# Autodesk Inventor assembly: Additional_Building
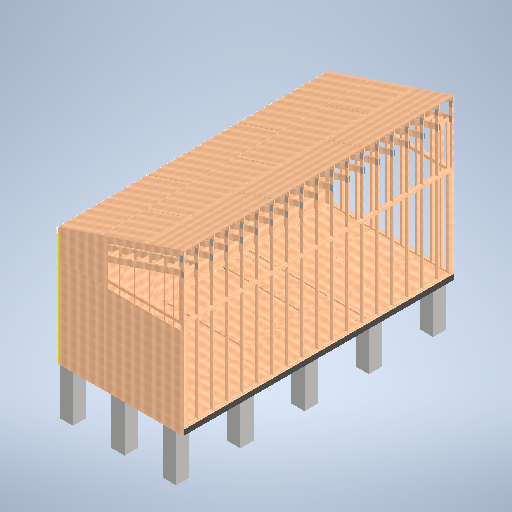
[picture p0: Inventor's stored thumbnail of the model, 512x512]
Saved by Autodesk Inventor 2025 (Build 290162010, 162A)
## iProperties
Created: 2024-08-02
Part Number: Additional_Building
Document SubType Name: Assembly
Designer: Tom
Author: Tom
## Documents named in this file (35)
- C:\Users\Tom\Documents\Inventor\Mobility\Additional_Building\Additional_Building.iam
- C:\Users\Tom\Documents\Inventor\Mobility\Additional_Building\Grid_Of_Piers.iam
- C:\Users\Tom\Documents\Inventor\Mobility\Additional_Building\Floor_System.iam
- C:\Users\Tom\Documents\Inventor\Mobility\Additional_Building\Walls.iam
- C:\Users\Tom\Documents\Inventor\Mobility\Additional_Building\Truss.iam
- C:\Users\Tom\Documents\Inventor\Mobility\Additional_Building\OSB_For_Walls_With_Dimensions_48_x_96_Inches.ipt
- C:\Users\Tom\Documents\Inventor\Mobility\Additional_Building\OSB_For_Walls_With_Dimensions_48_x_48_Inches.ipt
- C:\Users\Tom\Documents\Inventor\Mobility\Additional_Building\OSB_For_Roof_With_Dimensions_96_x_48.ipt
- C:\Users\Tom\Documents\Inventor\Mobility\Additional_Building\OSB_For_Walls_With_Dimensions_25.5_x_96_Inches.ipt
- C:\Users\Tom\Documents\Inventor\Mobility\Additional_Building\Subfascia_With_Width_13.75_Inches.ipt
- C:\Users\Tom\Documents\Inventor\Mobility\Additional_Building\Subfascia_With_Width_14.5_Inches.ipt
- C:\Users\Tom\Documents\Inventor\Mobility\Additional_Building\DensGlass_With_Dimensions_36.5_x_48_Inches.ipt
- C:\Users\Tom\Documents\Inventor\Mobility\Additional_Building\DensGlass_With_Dimensions_48_x_96_Inches.ipt
- C:\Users\Tom\Documents\Inventor\Mobility\Additional_Building\DensGlass_With_Dimensions_48_x_84.5_Inches.ipt
- C:\Users\Tom\Documents\Inventor\Mobility\Additional_Building\DensGlass_With_Dimensions_60.75_x_12_Inches.ipt
- C:\Users\Tom\Documents\Inventor\Mobility\Additional_Building\DensGlass_With_Dimensions_36.5_x_25.5_Inches.ipt
- C:\Users\Tom\Documents\Inventor\Mobility\Additional_Building\DensGlass_With_Dimensions_25.5_x_96_Inches.ipt
- C:\Users\Tom\Documents\Inventor\Mobility\Additional_Building\Siding_For_Back_Wall.iam
- C:\Users\Tom\Documents\Inventor\Mobility\Additional_Building\Fascia.ipt
- C:\Users\Tom\Documents\Inventor\Mobility\Additional_Building\OSB_For_Walls_With_Dimensions_37_x_96_Inches.ipt
- C:\Users\Tom\Documents\Inventor\Mobility\Additional_Building\OSB_For_Side_And_Back.ipt
- C:\Users\Tom\Documents\Inventor\Mobility\Additional_Building\Siding_For_Side_Wall.iam
- C:\Users\Tom\Documents\Inventor\Mobility\Additional_Building\OSB_For_Roof_With_Dimensions_48_x_48.ipt
- C:\Users\Tom\Documents\Inventor\Mobility\Additional_Building\OSB_For_Roof_With_Dimensions_45.796_x_48.ipt
- C:\Users\Tom\Documents\Inventor\Mobility\Additional_Building\Stud_Between_Top_Plate_And_Rafter_1.ipt
- C:\Users\Tom\Documents\Inventor\Mobility\Additional_Building\Stud_Between_Top_Plate_And_Rafter_2.ipt
- C:\Users\Tom\Documents\Inventor\Mobility\Additional_Building\Stud_Between_Top_Plate_And_Rafter_3.ipt
- C:\Users\Tom\Documents\Inventor\Mobility\Additional_Building\Stud_Between_Top_Plate_And_Rafter_4.ipt
- C:\Users\Tom\Documents\Inventor\Mobility\Additional_Building\Stud_Between_Top_Plate_And_Rafter_5.ipt
- C:\Users\Tom\Documents\Inventor\Mobility\Additional_Building\Stud_Between_Top_Plate_And_Rafter_6.ipt
- C:\Users\Tom\Documents\Inventor\Mobility\Additional_Building\Stud_Between_Top_Plate_And_Rafter_7.ipt
- C:\Users\Tom\Documents\Inventor\Mobility\Additional_Building\Stud_Between_Top_Plate_And_Rafter_8.ipt
- C:\Users\Tom\Documents\Inventor\Mobility\Additional_Building\Stud_Between_Top_Plate_And_Rafter_9.ipt
- C:\Users\Tom\Documents\Inventor\Mobility\Additional_Building\Stud_With_Height_41.707_Inches.ipt
- C:\Users\Tom\Documents\Inventor\Mobility\Additional_Building\Support_For_Ceiling.ipt
## Components (124 placed, 34 different names)
1. Grid_Of_Piers:1 [sub-assembly] — Mate:1, Flush:1, Mate:2
2. Floor_System:1 [sub-assembly] — Mate:1, Flush:1, Mate:2, Mate:3, Flush:2, Flush:3, Flush:15, Flush:16, Flush:29, Flush:30, Flush:31, Flush:33, Mate:51, Flush:41, Mate:53, Flush:42, Mate:55, Flush:44
3. Walls:1 [sub-assembly] — Mate:3, Flush:2, Flush:3, Flush:4, Flush:5, Mate:4, Flush:7, Mate:5, Mate:9, Mate:10, Flush:17, Mate:12, Mate:15, Mate:18, Mate:68, Flush:48, Flush:49, Mate:69, Flush:50, Flush:51, Mate:70, Flush:52, Flush:53, Mate:71, Flush:54, Flush:55, Mate:72, Flush:56, Flush:57, Mate:73, Flush:58, Flush:59, Mate:74, Flush:60, Flush:61, Mate:75, Flush:62, Flush:63, Mate:76, Flush:64, Mate:78, Mate:90
4. OSB_For_Walls_With_Dimensions_48_x_48_Inches:1 — Mate:10, Mate:11, Flush:17, Mate:13, Mate:34
5. OSB_For_Walls_With_Dimensions_48_x_48_Inches:2 — Mate:15, Mate:16, Mate:17, Mate:29, Flush:32
6. Subfascia_With_Width_13.75_Inches:1 — Mate:21, Flush:22, Flush:23
7. Subfascia_With_Width_13.75_Inches:2 — Flush:26, Mate:23, Flush:27, Flush:39
8. DensGlass_With_Dimensions_36.5_x_48_Inches:1 — Mate:24, Flush:28, Flush:29, Mate:26
9. DensGlass_With_Dimensions_36.5_x_48_Inches:2 — Mate:27, Mate:28, Flush:31
10. DensGlass_With_Dimensions_48_x_84.5_Inches:1 — Mate:29, Flush:32, Mate:30, Mate:32, Mate:38, Mate:41, Mate:44
11. DensGlass_With_Dimensions_48_x_96_Inches:3 — Mate:31, Mate:32, Mate:33, Mate:35
12. DensGlass_With_Dimensions_48_x_84.5_Inches:2 — Mate:34, Mate:35, Mate:36, Mate:47
13. DensGlass_With_Dimensions_36.5_x_25.5_Inches:1 — Mate:39, Mate:40, Mate:41, Mate:43
14. DensGlass_With_Dimensions_36.5_x_25.5_Inches:2 — Mate:45, Mate:46, Mate:47
15. Siding_For_Back_Wall:1 [sub-assembly] — Mate:48, Flush:34, Flush:35
16. OSB_For_Walls_With_Dimensions_48_x_96_Inches:6 — Mate:51, Mate:52, Flush:41, Mate:54, Mate:58, Mate:59
17. OSB_For_Walls_With_Dimensions_48_x_96_Inches:7 — Mate:53, Mate:54, Flush:42, Mate:93
18. OSB_For_Walls_With_Dimensions_37_x_96_Inches:1 — Mate:55, Flush:44, Flush:45, Mate:93
19. OSB_For_Side_And_Back:1 — Mate:56, Mate:57, Mate:58
20. Siding_For_Side_Wall:1 [sub-assembly] — Mate:59, Mate:60, Flush:45
21. Truss:1 [sub-assembly] — Flush:6, Mate:23, Flush:27, Mate:50, Flush:40, Mate:56, Mate:77, Mate:79, Flush:65, Flush:67, Flush:69, Flush:71, Flush:73, Flush:75, Flush:77, Flush:79, Flush:81, Mate:92
22. Truss:2 [sub-assembly] — Flush:4, Flush:5, Mate:4, Mate:20, Mate:49, Flush:36, Flush:37, Mate:62, Mate:66
23. Truss:3 [sub-assembly] — Flush:6, Flush:7, Mate:5, Flush:26, Mate:81, Mate:82, Mate:83, Mate:84, Mate:85, Mate:86, Mate:87, Mate:88, Mate:89, Mate:91, Flush:82
24. Truss:4 [sub-assembly]
25. Truss:5 [sub-assembly]
26. Truss:6 [sub-assembly]
27. Truss:7 [sub-assembly]
28. Truss:8 [sub-assembly]
29. Truss:9 [sub-assembly]
30. Truss:10 [sub-assembly]
31. Truss:11 [sub-assembly]
32. Truss:12 [sub-assembly]
33. Truss:13 [sub-assembly]
34. Truss:14 [sub-assembly]
35. Truss:15 [sub-assembly] — Mate:63
36. Truss:16 [sub-assembly]
37. Truss:17 [sub-assembly]
38. Truss:18 [sub-assembly] — Mate:22, Flush:25
39. Truss:19 [sub-assembly] — Mate:21, Flush:22, Flush:23, Flush:24
40. OSB_For_Roof_With_Dimensions_96_x_48:1
41. OSB_For_Roof_With_Dimensions_96_x_48:2 — Mate:64
42. OSB_For_Roof_With_Dimensions_96_x_48:3 — Mate:49, Flush:36, Flush:37, Mate:61, Flush:46
43. OSB_For_Roof_With_Dimensions_48_x_48:1 — Mate:61, Mate:62, Flush:46, Mate:65, Mate:67, Flush:47
44. OSB_For_Roof_With_Dimensions_48_x_48:2
45. OSB_For_Roof_With_Dimensions_96_x_48:4 — Mate:63, Mate:64, Mate:65
46. OSB_For_Roof_With_Dimensions_96_x_48:5
47. OSB_For_Roof_With_Dimensions_45.796_x_48:1 — Mate:66, Mate:67, Flush:47
48. OSB_For_Roof_With_Dimensions_45.796_x_48:2
49. OSB_For_Roof_With_Dimensions_45.796_x_48:3
50. OSB_For_Walls_With_Dimensions_48_x_96_Inches:1 — Mate:9, Flush:15, Flush:16, Mate:11, Mate:16, Flush:18, Mate:24, Flush:28, Mate:25, Mate:37
51. OSB_For_Walls_With_Dimensions_48_x_96_Inches:2
52. OSB_For_Walls_With_Dimensions_48_x_96_Inches:3 — Mate:14, Mate:27
53. OSB_For_Walls_With_Dimensions_48_x_96_Inches:4 — Mate:12, Mate:13, Mate:14, Mate:31
54. OSB_For_Walls_With_Dimensions_48_x_96_Inches:5 — Mate:17
55. OSB_For_Walls_With_Dimensions_25.5_x_96_Inches:1 — Mate:18, Flush:18, Mate:20, Mate:39
56. OSB_For_Walls_With_Dimensions_25.5_x_96_Inches:2 — Mate:42
57. OSB_For_Walls_With_Dimensions_25.5_x_96_Inches:3 — Mate:45
58. Subfascia_With_Width_14.5_Inches:1 — Flush:24, Mate:22, Flush:25
59. Subfascia_With_Width_14.5_Inches:2
60. Subfascia_With_Width_14.5_Inches:3
61. Subfascia_With_Width_14.5_Inches:4
62. Subfascia_With_Width_14.5_Inches:5
63. Subfascia_With_Width_14.5_Inches:6
64. Subfascia_With_Width_14.5_Inches:7
65. Subfascia_With_Width_14.5_Inches:8
66. Subfascia_With_Width_14.5_Inches:9
67. Subfascia_With_Width_14.5_Inches:10
68. Subfascia_With_Width_14.5_Inches:11
69. Subfascia_With_Width_14.5_Inches:12
70. Subfascia_With_Width_14.5_Inches:13
71. Subfascia_With_Width_14.5_Inches:14
72. Subfascia_With_Width_14.5_Inches:15
73. Subfascia_With_Width_14.5_Inches:16
74. DensGlass_With_Dimensions_48_x_96_Inches:1 — Mate:25, Mate:26, Flush:30, Mate:30, Mate:33
75. DensGlass_With_Dimensions_48_x_96_Inches:2 — Mate:28, Mate:36
76. DensGlass_With_Dimensions_60.75_x_12_Inches:1 — Mate:37, Mate:38, Flush:33
77. DensGlass_With_Dimensions_60.75_x_12_Inches:2 — Mate:48, Flush:34, Flush:35, Mate:52
78. DensGlass_With_Dimensions_60.75_x_12_Inches:3 — Mate:40
79. DensGlass_With_Dimensions_60.75_x_12_Inches:4 — Mate:57
80. DensGlass_With_Dimensions_25.5_x_96_Inches:1 — Mate:42, Mate:43, Mate:44
81. DensGlass_With_Dimensions_25.5_x_96_Inches:2 — Mate:46
82. Fascia:1 — Mate:50, Flush:39, Flush:40, Mate:60
83. Fascia:2
84. Fascia:3
85. Stud_Between_Top_Plate_And_Rafter_1:1 — Mate:68, Flush:48, Flush:49, Flush:66
86. Stud_Between_Top_Plate_And_Rafter_2:1 — Mate:69, Flush:50, Flush:51, Flush:68
87. Stud_Between_Top_Plate_And_Rafter_3:1 — Mate:70, Flush:52, Flush:53, Flush:70
88. Stud_Between_Top_Plate_And_Rafter_4:1 — Mate:71, Flush:54, Flush:55, Flush:72
89. Stud_Between_Top_Plate_And_Rafter_5:1 — Mate:72, Flush:56, Flush:57, Flush:74
90. Stud_Between_Top_Plate_And_Rafter_6:1 — Mate:73, Flush:58, Flush:59, Flush:76
91. Stud_Between_Top_Plate_And_Rafter_7:1 — Mate:74, Flush:60, Flush:61, Flush:78
92. Stud_Between_Top_Plate_And_Rafter_9:1 — Mate:76, Mate:77, Flush:64, Mate:80
93. Stud_Between_Top_Plate_And_Rafter_8:1 — Mate:75, Flush:62, Flush:63, Flush:80
94. Stud_Between_Top_Plate_And_Rafter_1:2
95. Stud_Between_Top_Plate_And_Rafter_2:2
96. Stud_Between_Top_Plate_And_Rafter_3:2
97. Stud_Between_Top_Plate_And_Rafter_4:2
98. Stud_Between_Top_Plate_And_Rafter_5:2
99. Stud_Between_Top_Plate_And_Rafter_6:2
100. Stud_Between_Top_Plate_And_Rafter_7:2
101. Stud_Between_Top_Plate_And_Rafter_9:2
102. Stud_Between_Top_Plate_And_Rafter_8:2
103. Stud_With_Height_41.707_Inches:1 — Mate:78, Mate:79, Mate:80
104. Stud_With_Height_41.707_Inches:2
105. Support_For_Ceiling:9 — Mate:89, Flush:81, Mate:90
106. Support_For_Ceiling:1 — Mate:81, Flush:65, Flush:66
107. Support_For_Ceiling:2 — Mate:82, Flush:67, Flush:68
108. Support_For_Ceiling:3 — Mate:83, Flush:69, Flush:70
109. Support_For_Ceiling:4 — Mate:84, Flush:71, Flush:72
110. Support_For_Ceiling:5 — Mate:85, Flush:73, Flush:74
111. Support_For_Ceiling:6 — Mate:86, Flush:75, Flush:76
112. Support_For_Ceiling:7 — Mate:87, Flush:77, Flush:78
113. Support_For_Ceiling:8 — Mate:88, Flush:79, Flush:80
114. Support_For_Ceiling:10 — Mate:91, Flush:82, Mate:92
115. Support_For_Ceiling:11
116. Support_For_Ceiling:12
117. Support_For_Ceiling:13
118. Support_For_Ceiling:14
119. Support_For_Ceiling:15
120. Support_For_Ceiling:16
121. Support_For_Ceiling:17
122. Support_For_Ceiling:18
123. Support_For_Ceiling:19
124. Support_For_Ceiling:20
## Component patterns: (2 elements, first: Truss:1), (17 elements, first: Truss:3), (3 elements, first: OSB_For_Roof_With_Dimensions_96_x_48:1), (2 elements, first: OSB_For_Roof_With_Dimensions_48_x_48:1), (2 elements, first: OSB_For_Roof_With_Dimensions_96_x_48:4), (3 elements, first: OSB_For_Roof_With_Dimensions_45.796_x_48:1), (3 elements, first: OSB_For_Walls_With_Dimensions_48_x_96_Inches:1), (2 elements, first: OSB_For_Walls_With_Dimensions_48_x_96_Inches:4), (3 elements, first: OSB_For_Walls_With_Dimensions_25.5_x_96_Inches:1), (16 elements, first: Subfascia_With_Width_14.5_Inches:1), (2 elements, first: DensGlass_With_Dimensions_48_x_96_Inches:1), (4 elements, first: DensGlass_With_Dimensions_60.75_x_12_Inches:1), (2 elements, first: DensGlass_With_Dimensions_25.5_x_96_Inches:1), (3 elements, first: Fascia:1), (2 elements, first: Stud_Between_Top_Plate_And_Rafter_1:1 + Stud_Between_Top_Plate_And_Rafter_2:1 + Stud_Between_Top_Plate_And_Rafter_3:1 + Stud_Between_Top_Plate_And_Rafter_4:1 + Stud_Between_Top_Plate_And_Rafter_5:1 + Stud_Between_Top_Plate_And_Rafter_6:1 + Stud_Between_Top_Plate_And_Rafter_7:1 + Stud_Between_Top_Plate_And_Rafter_9:1 + Stud_Between_Top_Plate_And_Rafter_8:1), (2 elements, first: Stud_With_Height_41.707_Inches:1), (2 elements, first: Support_For_Ceiling:9 + Support_For_Ceiling:1 + Support_For_Ceiling:2 + Support_For_Ceiling:3 + Support_For_Ceiling:4 + Support_For_Ceiling:5 + Support_For_Ceiling:6 + Support_For_Ceiling:7 + Support_For_Ceiling:8 + Support_For_Ceiling:10)
## Relationships (159: Mate 89, Flush 70)
- Mate:1: Grid_Of_Piers:1 ↔ Floor_System:1
- Flush:1: Grid_Of_Piers:1 ↔ Floor_System:1
- Mate:2: Grid_Of_Piers:1 ↔ Floor_System:1
- Mate:3: Floor_System:1 ↔ Walls:1
- Flush:2: Floor_System:1 ↔ Walls:1
- Flush:3: Floor_System:1 ↔ Walls:1
- Flush:4: Walls:1 ↔ Truss:2
- Flush:5: Walls:1 ↔ Truss:2
- Mate:4: Walls:1 ↔ Truss:2
- Flush:6 (387.35 mm): Truss:1 ↔ Truss:3
- Flush:7: Walls:1 ↔ Truss:3
- Mate:5: Walls:1 ↔ Truss:3
- Mate:9: Walls:1 ↔ OSB_For_Walls_With_Dimensions_48_x_96_Inches:1
- Flush:15: Floor_System:1 ↔ OSB_For_Walls_With_Dimensions_48_x_96_Inches:1
- Flush:16: Floor_System:1 ↔ OSB_For_Walls_With_Dimensions_48_x_96_Inches:1
- Mate:10: Walls:1 ↔ OSB_For_Walls_With_Dimensions_48_x_48_Inches:1
- Mate:11: OSB_For_Walls_With_Dimensions_48_x_48_Inches:1 ↔ OSB_For_Walls_With_Dimensions_48_x_96_Inches:1
- Flush:17: Walls:1 ↔ OSB_For_Walls_With_Dimensions_48_x_48_Inches:1
- Mate:12: Walls:1 ↔ OSB_For_Walls_With_Dimensions_48_x_96_Inches:4
- Mate:13: OSB_For_Walls_With_Dimensions_48_x_48_Inches:1 ↔ OSB_For_Walls_With_Dimensions_48_x_96_Inches:4
- Mate:14: OSB_For_Walls_With_Dimensions_48_x_96_Inches:3 ↔ OSB_For_Walls_With_Dimensions_48_x_96_Inches:4
- Mate:15: Walls:1 ↔ OSB_For_Walls_With_Dimensions_48_x_48_Inches:2
- Mate:16: OSB_For_Walls_With_Dimensions_48_x_48_Inches:2 ↔ OSB_For_Walls_With_Dimensions_48_x_96_Inches:1
- Mate:17: OSB_For_Walls_With_Dimensions_48_x_48_Inches:2 ↔ OSB_For_Walls_With_Dimensions_48_x_96_Inches:5
- Mate:18: Walls:1 ↔ OSB_For_Walls_With_Dimensions_25.5_x_96_Inches:1
- Flush:18: OSB_For_Walls_With_Dimensions_48_x_96_Inches:1 ↔ OSB_For_Walls_With_Dimensions_25.5_x_96_Inches:1
- Mate:20: Truss:2 ↔ OSB_For_Walls_With_Dimensions_25.5_x_96_Inches:1
- Mate:21: Subfascia_With_Width_13.75_Inches:1 ↔ Truss:19
- Flush:22: Subfascia_With_Width_13.75_Inches:1 ↔ Truss:19
- Flush:23: Subfascia_With_Width_13.75_Inches:1 ↔ Truss:19
- Flush:24: Truss:19 ↔ Subfascia_With_Width_14.5_Inches:1
- Mate:22: Truss:18 ↔ Subfascia_With_Width_14.5_Inches:1
- Flush:25: Truss:18 ↔ Subfascia_With_Width_14.5_Inches:1
- Flush:26: Subfascia_With_Width_13.75_Inches:2 ↔ Truss:3
- Mate:23: Subfascia_With_Width_13.75_Inches:2 ↔ Truss:1
- Flush:27: Subfascia_With_Width_13.75_Inches:2 ↔ Truss:1
- Mate:24: DensGlass_With_Dimensions_36.5_x_48_Inches:1 ↔ OSB_For_Walls_With_Dimensions_48_x_96_Inches:1
- Flush:28 (292.1 mm): DensGlass_With_Dimensions_36.5_x_48_Inches:1 ↔ OSB_For_Walls_With_Dimensions_48_x_96_Inches:1
- Flush:29: Floor_System:1 ↔ DensGlass_With_Dimensions_36.5_x_48_Inches:1
- Mate:25: OSB_For_Walls_With_Dimensions_48_x_96_Inches:1 ↔ DensGlass_With_Dimensions_48_x_96_Inches:1
- Mate:26: DensGlass_With_Dimensions_36.5_x_48_Inches:1 ↔ DensGlass_With_Dimensions_48_x_96_Inches:1
- Flush:30: Floor_System:1 ↔ DensGlass_With_Dimensions_48_x_96_Inches:1
- Mate:27: DensGlass_With_Dimensions_36.5_x_48_Inches:2 ↔ OSB_For_Walls_With_Dimensions_48_x_96_Inches:3
- Mate:28: DensGlass_With_Dimensions_36.5_x_48_Inches:2 ↔ DensGlass_With_Dimensions_48_x_96_Inches:2
- Flush:31: Floor_System:1 ↔ DensGlass_With_Dimensions_36.5_x_48_Inches:2
- Mate:29: OSB_For_Walls_With_Dimensions_48_x_48_Inches:2 ↔ DensGlass_With_Dimensions_48_x_84.5_Inches:1
- Flush:32 (292.1 mm): OSB_For_Walls_With_Dimensions_48_x_48_Inches:2 ↔ DensGlass_With_Dimensions_48_x_84.5_Inches:1
- Mate:30: DensGlass_With_Dimensions_48_x_84.5_Inches:1 ↔ DensGlass_With_Dimensions_48_x_96_Inches:1
- Mate:31: DensGlass_With_Dimensions_48_x_96_Inches:3 ↔ OSB_For_Walls_With_Dimensions_48_x_96_Inches:4
- Mate:32: DensGlass_With_Dimensions_48_x_84.5_Inches:1 ↔ DensGlass_With_Dimensions_48_x_96_Inches:3
- Mate:33: DensGlass_With_Dimensions_48_x_96_Inches:3 ↔ DensGlass_With_Dimensions_48_x_96_Inches:1
- Mate:34: OSB_For_Walls_With_Dimensions_48_x_48_Inches:1 ↔ DensGlass_With_Dimensions_48_x_84.5_Inches:2
- Mate:35: DensGlass_With_Dimensions_48_x_96_Inches:3 ↔ DensGlass_With_Dimensions_48_x_84.5_Inches:2
- Mate:36: DensGlass_With_Dimensions_48_x_84.5_Inches:2 ↔ DensGlass_With_Dimensions_48_x_96_Inches:2
- Mate:37: OSB_For_Walls_With_Dimensions_48_x_96_Inches:1 ↔ DensGlass_With_Dimensions_60.75_x_12_Inches:1
- Mate:38: DensGlass_With_Dimensions_48_x_84.5_Inches:1 ↔ DensGlass_With_Dimensions_60.75_x_12_Inches:1
- Flush:33: Floor_System:1 ↔ DensGlass_With_Dimensions_60.75_x_12_Inches:1
- Mate:39: DensGlass_With_Dimensions_36.5_x_25.5_Inches:1 ↔ OSB_For_Walls_With_Dimensions_25.5_x_96_Inches:1
- Mate:40: DensGlass_With_Dimensions_36.5_x_25.5_Inches:1 ↔ DensGlass_With_Dimensions_60.75_x_12_Inches:3
- Mate:41: DensGlass_With_Dimensions_48_x_84.5_Inches:1 ↔ DensGlass_With_Dimensions_36.5_x_25.5_Inches:1
- Mate:42: OSB_For_Walls_With_Dimensions_25.5_x_96_Inches:2 ↔ DensGlass_With_Dimensions_25.5_x_96_Inches:1
- Mate:43: DensGlass_With_Dimensions_36.5_x_25.5_Inches:1 ↔ DensGlass_With_Dimensions_25.5_x_96_Inches:1
- Mate:44: DensGlass_With_Dimensions_48_x_84.5_Inches:1 ↔ DensGlass_With_Dimensions_25.5_x_96_Inches:1
- Mate:45: DensGlass_With_Dimensions_36.5_x_25.5_Inches:2 ↔ OSB_For_Walls_With_Dimensions_25.5_x_96_Inches:3
- Mate:46: DensGlass_With_Dimensions_36.5_x_25.5_Inches:2 ↔ DensGlass_With_Dimensions_25.5_x_96_Inches:2
- Mate:47: DensGlass_With_Dimensions_48_x_84.5_Inches:2 ↔ DensGlass_With_Dimensions_36.5_x_25.5_Inches:2
- Mate:48: Siding_For_Back_Wall:1 ↔ DensGlass_With_Dimensions_60.75_x_12_Inches:2
- Flush:34: Siding_For_Back_Wall:1 ↔ DensGlass_With_Dimensions_60.75_x_12_Inches:2
- Flush:35: Siding_For_Back_Wall:1 ↔ DensGlass_With_Dimensions_60.75_x_12_Inches:2
- Mate:49: Truss:2 ↔ OSB_For_Roof_With_Dimensions_96_x_48:3
- Flush:36: Truss:2 ↔ OSB_For_Roof_With_Dimensions_96_x_48:3
- Flush:37: Truss:2 ↔ OSB_For_Roof_With_Dimensions_96_x_48:3
- Mate:50: Truss:1 ↔ Fascia:1
- Flush:39 (-12.319 mm): Subfascia_With_Width_13.75_Inches:2 ↔ Fascia:1
- Flush:40 (-30.3276 mm): Truss:1 ↔ Fascia:1
- Mate:51: Floor_System:1 ↔ OSB_For_Walls_With_Dimensions_48_x_96_Inches:6
- Mate:52: OSB_For_Walls_With_Dimensions_48_x_96_Inches:6 ↔ DensGlass_With_Dimensions_60.75_x_12_Inches:2
- Flush:41: Floor_System:1 ↔ OSB_For_Walls_With_Dimensions_48_x_96_Inches:6
- Mate:53: Floor_System:1 ↔ OSB_For_Walls_With_Dimensions_48_x_96_Inches:7
- Mate:54: OSB_For_Walls_With_Dimensions_48_x_96_Inches:6 ↔ OSB_For_Walls_With_Dimensions_48_x_96_Inches:7
- Flush:42: Floor_System:1 ↔ OSB_For_Walls_With_Dimensions_48_x_96_Inches:7
- Mate:55: Floor_System:1 ↔ OSB_For_Walls_With_Dimensions_37_x_96_Inches:1
- Flush:44: Floor_System:1 ↔ OSB_For_Walls_With_Dimensions_37_x_96_Inches:1
- Mate:56: OSB_For_Side_And_Back:1 ↔ Truss:1
- Mate:57: OSB_For_Side_And_Back:1 ↔ DensGlass_With_Dimensions_60.75_x_12_Inches:4
- Mate:58: OSB_For_Walls_With_Dimensions_48_x_96_Inches:6 ↔ OSB_For_Side_And_Back:1
- Mate:59: OSB_For_Walls_With_Dimensions_48_x_96_Inches:6 ↔ Siding_For_Side_Wall:1
- Mate:60: Siding_For_Side_Wall:1 ↔ Fascia:1
- Flush:45 (-6.35 mm): OSB_For_Walls_With_Dimensions_37_x_96_Inches:1 ↔ Siding_For_Side_Wall:1
- Mate:61: OSB_For_Roof_With_Dimensions_96_x_48:3 ↔ OSB_For_Roof_With_Dimensions_48_x_48:1
- Mate:62: Truss:2 ↔ OSB_For_Roof_With_Dimensions_48_x_48:1
- Flush:46: OSB_For_Roof_With_Dimensions_96_x_48:3 ↔ OSB_For_Roof_With_Dimensions_48_x_48:1
- Mate:63: Truss:15 ↔ OSB_For_Roof_With_Dimensions_96_x_48:4
- Mate:64: OSB_For_Roof_With_Dimensions_96_x_48:2 ↔ OSB_For_Roof_With_Dimensions_96_x_48:4
- Mate:65: OSB_For_Roof_With_Dimensions_48_x_48:1 ↔ OSB_For_Roof_With_Dimensions_96_x_48:4
- Mate:66: Truss:2 ↔ OSB_For_Roof_With_Dimensions_45.796_x_48:1
- Mate:67: OSB_For_Roof_With_Dimensions_48_x_48:1 ↔ OSB_For_Roof_With_Dimensions_45.796_x_48:1
- Flush:47: OSB_For_Roof_With_Dimensions_48_x_48:1 ↔ OSB_For_Roof_With_Dimensions_45.796_x_48:1
- Mate:68: Walls:1 ↔ Stud_Between_Top_Plate_And_Rafter_1:1
- Flush:48: Walls:1 ↔ Stud_Between_Top_Plate_And_Rafter_1:1
- Flush:49: Walls:1 ↔ Stud_Between_Top_Plate_And_Rafter_1:1
- Mate:69: Walls:1 ↔ Stud_Between_Top_Plate_And_Rafter_2:1
- Flush:50: Walls:1 ↔ Stud_Between_Top_Plate_And_Rafter_2:1
- Flush:51: Walls:1 ↔ Stud_Between_Top_Plate_And_Rafter_2:1
- Mate:70: Walls:1 ↔ Stud_Between_Top_Plate_And_Rafter_3:1
- Flush:52: Walls:1 ↔ Stud_Between_Top_Plate_And_Rafter_3:1
- Flush:53: Walls:1 ↔ Stud_Between_Top_Plate_And_Rafter_3:1
- Mate:71: Walls:1 ↔ Stud_Between_Top_Plate_And_Rafter_4:1
- Flush:54: Walls:1 ↔ Stud_Between_Top_Plate_And_Rafter_4:1
- Flush:55: Walls:1 ↔ Stud_Between_Top_Plate_And_Rafter_4:1
- Mate:72: Walls:1 ↔ Stud_Between_Top_Plate_And_Rafter_5:1
- Flush:56: Walls:1 ↔ Stud_Between_Top_Plate_And_Rafter_5:1
- Flush:57: Walls:1 ↔ Stud_Between_Top_Plate_And_Rafter_5:1
- Mate:73: Walls:1 ↔ Stud_Between_Top_Plate_And_Rafter_6:1
- Flush:58: Walls:1 ↔ Stud_Between_Top_Plate_And_Rafter_6:1
- Flush:59: Walls:1 ↔ Stud_Between_Top_Plate_And_Rafter_6:1
- Mate:74: Walls:1 ↔ Stud_Between_Top_Plate_And_Rafter_7:1
- Flush:60: Walls:1 ↔ Stud_Between_Top_Plate_And_Rafter_7:1
- Flush:61: Walls:1 ↔ Stud_Between_Top_Plate_And_Rafter_7:1
- Mate:75: Walls:1 ↔ Stud_Between_Top_Plate_And_Rafter_8:1
- Flush:62: Walls:1 ↔ Stud_Between_Top_Plate_And_Rafter_8:1
- Flush:63: Walls:1 ↔ Stud_Between_Top_Plate_And_Rafter_8:1
- Mate:76: Walls:1 ↔ Stud_Between_Top_Plate_And_Rafter_9:1
- Mate:77: Truss:1 ↔ Stud_Between_Top_Plate_And_Rafter_9:1
- Flush:64: Walls:1 ↔ Stud_Between_Top_Plate_And_Rafter_9:1
- Mate:78: Walls:1 ↔ Stud_With_Height_41.707_Inches:1
- Mate:79: Truss:1 ↔ Stud_With_Height_41.707_Inches:1
- Mate:80: Stud_Between_Top_Plate_And_Rafter_9:1 ↔ Stud_With_Height_41.707_Inches:1
- Mate:81: Truss:3 ↔ Support_For_Ceiling:1
- Flush:65: Truss:1 ↔ Support_For_Ceiling:1
- Flush:66: Stud_Between_Top_Plate_And_Rafter_1:1 ↔ Support_For_Ceiling:1
- Mate:82: Truss:3 ↔ Support_For_Ceiling:2
- Flush:67: Truss:1 ↔ Support_For_Ceiling:2
- Flush:68: Stud_Between_Top_Plate_And_Rafter_2:1 ↔ Support_For_Ceiling:2
- Mate:83: Truss:3 ↔ Support_For_Ceiling:3
- Flush:69: Truss:1 ↔ Support_For_Ceiling:3
- Flush:70: Stud_Between_Top_Plate_And_Rafter_3:1 ↔ Support_For_Ceiling:3
- Mate:84: Truss:3 ↔ Support_For_Ceiling:4
- Flush:71: Truss:1 ↔ Support_For_Ceiling:4
- Flush:72: Stud_Between_Top_Plate_And_Rafter_4:1 ↔ Support_For_Ceiling:4
- Mate:85: Truss:3 ↔ Support_For_Ceiling:5
- Flush:73: Truss:1 ↔ Support_For_Ceiling:5
- Flush:74: Stud_Between_Top_Plate_And_Rafter_5:1 ↔ Support_For_Ceiling:5
- Mate:86: Truss:3 ↔ Support_For_Ceiling:6
- Flush:75: Truss:1 ↔ Support_For_Ceiling:6
- Flush:76: Stud_Between_Top_Plate_And_Rafter_6:1 ↔ Support_For_Ceiling:6
- Mate:87: Truss:3 ↔ Support_For_Ceiling:7
- Flush:77: Truss:1 ↔ Support_For_Ceiling:7
- Flush:78: Stud_Between_Top_Plate_And_Rafter_7:1 ↔ Support_For_Ceiling:7
- Mate:88: Truss:3 ↔ Support_For_Ceiling:8
- Flush:79: Truss:1 ↔ Support_For_Ceiling:8
- Flush:80: Stud_Between_Top_Plate_And_Rafter_8:1 ↔ Support_For_Ceiling:8
- Mate:89: Truss:3 ↔ Support_For_Ceiling:9
- Flush:81: Truss:1 ↔ Support_For_Ceiling:9
- Mate:90: Walls:1 ↔ Support_For_Ceiling:9
- Mate:91: Truss:3 ↔ Support_For_Ceiling:10
- Flush:82: Truss:3 ↔ Support_For_Ceiling:10
- Mate:92: Truss:1 ↔ Support_For_Ceiling:10
- Mate:93: OSB_For_Walls_With_Dimensions_48_x_96_Inches:7 ↔ OSB_For_Walls_With_Dimensions_37_x_96_Inches:1
